# Autodesk Inventor assembly: 2456K220_MIL. SPEC. PIN-AND-BLOCK U-JOINT
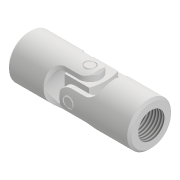
[picture p0: Inventor's stored thumbnail of the model, 180x180]
Saved by Autodesk Inventor 2021 (Build 250183000, 183)
## iProperties
Created: 2021-08-20
Part Number: 2456K220_MIL. SPEC. PIN-AND-BLOCK U-JOINT
Document SubType Name: Assembly
Designer: Santiago Suárez
Author: Santiago Suárez
## Documents named in this file (5)
- C:\Users\Santiago Suárez\Documents\GitHub\Dis.-Mecatronico-E6\inventor proyecto\cardan\2456K220_MIL. SPEC. PIN-AND-BLOCK U-JOINT.iam
- C:\Users\Santiago Suárez\Documents\GitHub\Dis.-Mecatronico-E6\inventor proyecto\cardan\Solid4.ipt
- C:\Users\Santiago Suárez\Documents\GitHub\Dis.-Mecatronico-E6\inventor proyecto\cardan\Solid3.ipt
- C:\Users\Santiago Suárez\Documents\GitHub\Dis.-Mecatronico-E6\inventor proyecto\cardan\Solid2.ipt
- C:\Users\Santiago Suárez\Documents\GitHub\Dis.-Mecatronico-E6\inventor proyecto\cardan\Solid1.ipt
## Components (4 placed, 4 different names)
1. Solid4:1 — Rotational:1, Rotational:2, Rigid:1
2. Solid3:1 — Rigid:1
3. Solid2:1 — Rotational:2
4. Solid1:1 — Rotational:1
## Relationships (3: RevoluteJoint 2, WeldJoint 1)
- Rotational:1 [RevoluteJoint]: Solid4:1 ↔ Solid1:1
- Rotational:2 [RevoluteJoint]: Solid4:1 ↔ Solid2:1
- Rigid:1 [WeldJoint]: Solid4:1 ↔ Solid3:1
